# Autodesk Inventor assembly: CrazyCar
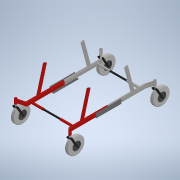
[picture p0: Inventor's stored thumbnail of the model, 180x180]
Saved by Autodesk Inventor 2022 (Build 260153000, 153)
## iProperties
Created: 2021-12-05
Part Number: CrazyCar
Document SubType Name: Assembly
Designer: Vedic
Author: Vedic
## Documents named in this file (10)
- C:\Users\hamen\Desktop\Everything Desktop\Inventor\CrazyCar\CrazyCar.iam
- C:\Users\hamen\Desktop\Everything Desktop\Inventor\CrazyCar\Liftarm.ipt
- C:\Users\hamen\Desktop\Everything Desktop\Inventor\CrazyCar\L-Bracket.ipt
- C:\Users\hamen\Desktop\Everything Desktop\Inventor\CrazyCar\Liftarm_MIR.ipt
- C:\Users\hamen\Desktop\Everything Desktop\Inventor\CrazyCar\Liftarm_MIR1.ipt
- C:\Users\hamen\Desktop\Everything Desktop\Inventor\CrazyCar\Liftarm_MIR_MIR.ipt
- C:\Users\hamen\Desktop\Everything Desktop\Inventor\CrazyCar\cross-beam.ipt
- C:\Users\hamen\Desktop\Everything Desktop\Inventor\CrazyCar\Wheel-Housing.ipt
- C:\Users\hamen\Desktop\Everything Desktop\Inventor\CrazyCar\wheel.ipt
- C:\Users\hamen\Desktop\Everything Desktop\Inventor\CrazyCar\0.375x1.0in Spacer.ipt
## Components (20 placed, 9 different names)
1. Liftarm:1 — Mate:8, Mate:11, Mate:12, Mate:21, Mate:22, Mate:23, Mate:35, Angle:1
2. L-Bracket:1 — Mate:2, Mate:3, Mate:4, Mate:5, Mate:6, Mate:7
3. L-Bracket:2 — Mate:8, Mate:9, Mate:10, Mate:11, Mate:12, Mate:13
4. Liftarm_MIR:1 — Mate:9, Mate:10, Mate:13, Mate:20, Mate:24, Mate:25, Mate:36, Angle:2
5. Liftarm_MIR1:1 — Mate:2, Mate:3, Mate:7, Mate:14, Mate:16, Mate:17, Mate:34, Mate:43, Angle:4
6. Liftarm_MIR_MIR:1 — Mate:4, Mate:5, Mate:6, Mate:15, Mate:18, Mate:19, Mate:37, Mate:38, Angle:3, Mate:72
7. cross-beam:1 — Mate:14, Mate:16, Mate:17, Mate:21, Mate:22, Mate:23
8. cross-beam:2 — Mate:15, Mate:18, Mate:19, Mate:20, Mate:24, Mate:25, Mate:72
9. Wheel-Housing:1 — Mate:26, Mate:27, Mate:34, Flush:1, Mate:40, Angle:4, Angle:6, Angle:7
10. wheel:1 — Mate:26, Mate:27
11. Wheel-Housing:2 — Mate:37, Flush:1, Flush:3, Mate:38, Mate:42, Angle:3, Angle:8
12. wheel:2
13. Wheel-Housing:3 — Mate:36, Flush:2, Flush:3, Mate:41, Angle:2, Angle:8, Angle:9
14. wheel:3
15. Wheel-Housing:4 — Mate:35, Flush:2, Mate:39, Angle:1, Flush:8, Angle:6, Angle:7, Angle:9
16. wheel:4
17. 0.375x1.0in Spacer:1 — Mate:39, Flush:4
18. 0.375x1.0in Spacer:2 — Mate:40, Flush:4, Flush:6, Mate:43
19. 0.375x1.0in Spacer:3 — Mate:42, Flush:5, Flush:6
20. 0.375x1.0in Spacer:4 — Mate:41, Flush:5
## Relationships (58: Mate 43, Angle 8, Flush 7)
- Mate:2: L-Bracket:1 ↔ Liftarm_MIR1:1
- Mate:3: L-Bracket:1 ↔ Liftarm_MIR1:1
- Mate:4: L-Bracket:1 ↔ Liftarm_MIR_MIR:1
- Mate:5: L-Bracket:1 ↔ Liftarm_MIR_MIR:1
- Mate:6: L-Bracket:1 ↔ Liftarm_MIR_MIR:1
- Mate:7: L-Bracket:1 ↔ Liftarm_MIR1:1
- Mate:8: Liftarm:1 ↔ L-Bracket:2
- Mate:9: L-Bracket:2 ↔ Liftarm_MIR:1
- Mate:10: L-Bracket:2 ↔ Liftarm_MIR:1
- Mate:11: Liftarm:1 ↔ L-Bracket:2
- Mate:12: Liftarm:1 ↔ L-Bracket:2
- Mate:13: L-Bracket:2 ↔ Liftarm_MIR:1
- Mate:14: Liftarm_MIR1:1 ↔ cross-beam:1
- Mate:15: Liftarm_MIR_MIR:1 ↔ cross-beam:2
- Mate:16: Liftarm_MIR1:1 ↔ cross-beam:1
- Mate:17: Liftarm_MIR1:1 ↔ cross-beam:1
- Mate:18: Liftarm_MIR_MIR:1 ↔ cross-beam:2
- Mate:19: Liftarm_MIR_MIR:1 ↔ cross-beam:2
- Mate:20: Liftarm_MIR:1 ↔ cross-beam:2
- Mate:21: Liftarm:1 ↔ cross-beam:1
- Mate:22: Liftarm:1 ↔ cross-beam:1
- Mate:23: Liftarm:1 ↔ cross-beam:1
- Mate:24: Liftarm_MIR:1 ↔ cross-beam:2
- Mate:25: Liftarm_MIR:1 ↔ cross-beam:2
- Mate:26: Wheel-Housing:1 ↔ wheel:1
- Mate:27: Wheel-Housing:1 ↔ wheel:1
- [Mate]: Wheel-Housing:2 ↔ wheel:2
- [Mate]: Wheel-Housing:2 ↔ wheel:2
- [Mate]: Wheel-Housing:3 ↔ wheel:3
- [Mate]: Wheel-Housing:3 ↔ wheel:3
- [Mate]: Wheel-Housing:4 ↔ wheel:4
- [Mate]: Wheel-Housing:4 ↔ wheel:4
- Mate:34: Liftarm_MIR1:1 ↔ Wheel-Housing:1
- Mate:35: Liftarm:1 ↔ Wheel-Housing:4
- Mate:36: Liftarm_MIR:1 ↔ Wheel-Housing:3
- Mate:37: Liftarm_MIR_MIR:1 ↔ Wheel-Housing:2
- Flush:1: Wheel-Housing:1 ↔ Wheel-Housing:2
- Flush:2: Wheel-Housing:3 ↔ Wheel-Housing:4
- Flush:3: Wheel-Housing:2 ↔ Wheel-Housing:3
- Mate:38 (25.4 mm): Liftarm_MIR_MIR:1 ↔ Wheel-Housing:2
- Mate:39: Wheel-Housing:4 ↔ 0.375x1.0in Spacer:1
- Mate:40: Wheel-Housing:1 ↔ 0.375x1.0in Spacer:2
- Mate:41: Wheel-Housing:3 ↔ 0.375x1.0in Spacer:4
- Mate:42: Wheel-Housing:2 ↔ 0.375x1.0in Spacer:3
- Flush:4: 0.375x1.0in Spacer:1 ↔ 0.375x1.0in Spacer:2
- Flush:5: 0.375x1.0in Spacer:3 ↔ 0.375x1.0in Spacer:4
- Flush:6: 0.375x1.0in Spacer:2 ↔ 0.375x1.0in Spacer:3
- Mate:43: Liftarm_MIR1:1 ↔ 0.375x1.0in Spacer:2
- Angle:1 (0 deg): Liftarm:1 ↔ Wheel-Housing:4
- Angle:2 (0 deg): Liftarm_MIR:1 ↔ Wheel-Housing:3
- Angle:3 (0 deg): Liftarm_MIR_MIR:1 ↔ Wheel-Housing:2
- Angle:4 (0 deg): Liftarm_MIR1:1 ↔ Wheel-Housing:1
- Mate:72: Liftarm_MIR_MIR:1 ↔ cross-beam:2
- Flush:8 (-209.8675 mm): Wheel-Housing:4
- Angle:6 (0 deg): Wheel-Housing:1 ↔ Wheel-Housing:4
- Angle:7 (0 deg): Wheel-Housing:1 ↔ Wheel-Housing:4
- Angle:8 (0 deg): Wheel-Housing:2 ↔ Wheel-Housing:3
- Angle:9 (0 deg): Wheel-Housing:3 ↔ Wheel-Housing:4
## Named parameters: d27_d25 = 0 mm, d28_d26 = 0 mm, d29_d25 = 0 mm, d30_d26 = 0 mm, d31_d25 = 0 mm, d32_d26 = 0 mm
